# Autodesk Inventor assembly: Shooter Mount6000
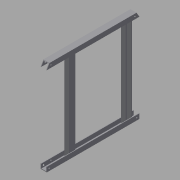
[picture p0: Inventor's stored thumbnail of the model, 180x180]
Saved by Autodesk Inventor 2013 (Build 170138000, 138)
## iProperties
Created: 2013-01-09
Part Number: Shooter Mount6000
Document SubType Name: Assembly
Designer: Naphat
Author: Naphat
## Documents named in this file (4)
- C:\Autodesk\gruntmaster6000-cad\Rack\Rack.iam
- C:\Autodesk\gruntmaster6000-cad\Rack\Rack - Back.ipt
- C:\Autodesk\gruntmaster6000-cad\Rack\Rack - Front.ipt
- C:\Autodesk\gruntmaster6000-cad\Rack\Rack - Cross Members.ipt
## Components (4 placed, 3 different names)
1. Rack - Back:1 — Mate:1, Mate:2, Mate:6, Mate:8
2. Rack - Front:1 — Mate:3, Mate:4, Insert:1, Mate:5
3. Rack - Cross Members:1 — Mate:5, Mate:6, Mate:7
4. Rack - Cross Members:2 — Mate:1, Mate:2, Mate:3, Mate:4, Insert:1, Mate:7, Mate:8
## Relationships (9: Mate 8, Insert 1)
- Mate:1: Rack - Back:1 ↔ Rack - Cross Members:2
- Mate:2: Rack - Back:1 ↔ Rack - Cross Members:2
- Mate:3: Rack - Front:1 ↔ Rack - Cross Members:2
- Mate:4: Rack - Front:1 ↔ Rack - Cross Members:2
- Insert:1: Rack - Front:1 ↔ Rack - Cross Members:2
- Mate:5: Rack - Front:1 ↔ Rack - Cross Members:1
- Mate:6: Rack - Back:1 ↔ Rack - Cross Members:1
- Mate:7 (264.5156 mm): Rack - Cross Members:1 ↔ Rack - Cross Members:2
- Mate:8: Rack - Back:1 ↔ Rack - Cross Members:2
